# Autodesk Inventor assembly: LegRightNCS
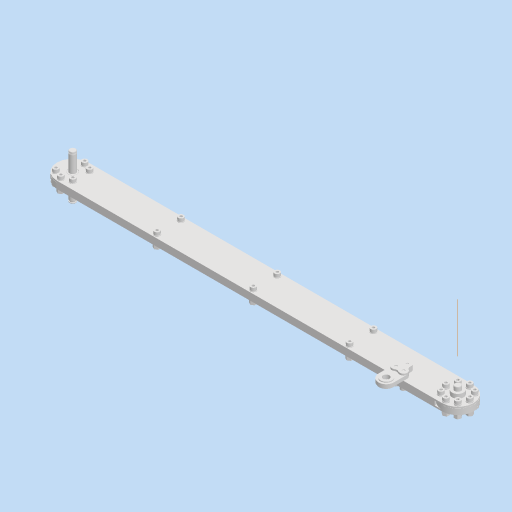
[picture p0: Inventor's stored thumbnail of the model, 512x512]
Saved by Autodesk Inventor 2023 (Build 270158000, 158)
## iProperties
Created: 2026-06-18
Part Number: LegRightNCS
Document SubType Name: Assembly
Designer: Nathann
Author: Nathann
## Documents named in this file (2)
- C:\Users\Nathann\ClawdDrive\Objet3D\RunningRobot\PartURDF\LegRightNCS.iam
- C:\Users\Nathann\ClawdDrive\Objet3D\RunningRobot\PartURDF\LegRight.iam
## Components (1 placed, 1 different names)
1. LegRight:1 [sub-assembly] — Mate:1, Flush:1, Flush:2, Flush:4, Flush:5
## Relationships (11: Flush 5, Mate 4, Symmetry 2)
- Mate:1: LegRight:1
- Mate:2
- Mate:3
- Flush:1: LegRight:1
- Flush:2: LegRight:1
- Symmetry:1
- Flush:3
- Flush:4: LegRight:1
- Flush:5: LegRight:1
- Symmetry:2
- Mate:4
